# Autodesk Inventor assembly: Robot_eslabones
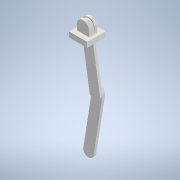
[picture p0: Inventor's stored thumbnail of the model, 180x180]
Saved by Autodesk Inventor 2021 (Build 250183000, 183)
## iProperties
Created: 2022-01-12
Part Number: Robot_eslabones
Document SubType Name: Assembly
Designer: Yeison
Author: Yeison
## Documents named in this file (5)
- C:\Users\Yeison\Documents\GitHub\Servomecanismos\Modelo 2021\Robot_eslabones.iam
- C:\Users\Yeison\Documents\GitHub\Servomecanismos\Modelo 2021\Soporte.ipt
- C:\Users\Yeison\Documents\GitHub\Servomecanismos\Modelo 2021\pin2.ipt
- C:\Users\Yeison\Documents\GitHub\Servomecanismos\Modelo 2021\Eslabon.ipt
- C:\Users\Yeison\Documents\GitHub\Servomecanismos\Modelo 2021\pin1.ipt
## Components (6 placed, 4 different names)
1. Soporte:1 — Rigid:1
2. pin2:1 — Rigid:1, Rotational:1
3. Eslabon:1 — Rotational:1, Rigid:2
4. pin2:2 — Rigid:2, Rotational:2
5. Eslabon:2 — Rotational:2, Rigid:3
6. pin1:1 — Rigid:3
## Relationships (5: WeldJoint 3, RevoluteJoint 2)
- Rigid:1 [WeldJoint]: Soporte:1 ↔ pin2:1
- Rotational:1 [RevoluteJoint]: pin2:1 ↔ Eslabon:1
- Rigid:2 [WeldJoint]: Eslabon:1 ↔ pin2:2
- Rotational:2 [RevoluteJoint] (-10 mm): pin2:2 ↔ Eslabon:2
- Rigid:3 [WeldJoint]: Eslabon:2 ↔ pin1:1
